# Autodesk Inventor assembly: Framework MASTER
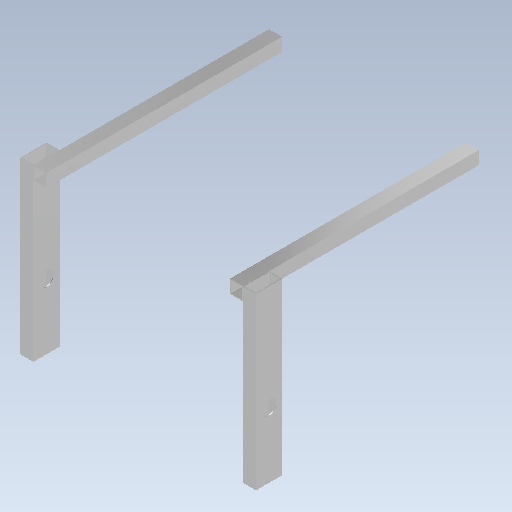
[picture p0: Inventor's stored thumbnail of the model, 512x512]
Saved by Autodesk Inventor 2020 (Build 240168000, 168)
## iProperties
Created: 2020-01-27
Part Number: Framework MASTER
Document SubType Name: Assembly
Designer: autum
Author: autum
## Documents named in this file (3)
- C:\Users\autum\Google Drive\Iron Riders 4180 (Roosevelt Robotics)\2019-2020\Build_Design\Robot 2020 (1)\Framework\Framework MASTER.iam
- C:\Users\autum\Google Drive\Iron Riders 4180 (Roosevelt Robotics)\2019-2020\Build_Design\Robot 2020 (1)\Framework\1x1 Top Frame.ipt
- C:\Users\autum\Google Drive\Iron Riders 4180 (Roosevelt Robotics)\2019-2020\Build_Design\Robot 2020 (1)\Framework\1x2 Frame.ipt
## Components (4 placed, 2 different names)
1. 1x1 Top Frame:1 — Mate:2, Flush:16, Flush:17
2. 1x1 Top Frame:2 — Flush:13, Flush:15, Mate:1
3. 1x2 Frame:1 — Flush:13, Flush:15, Mate:1
4. 1x2 Frame:2 — Mate:2, Flush:16, Flush:17
## Relationships (6: Flush 4, Mate 2)
- Flush:13: 1x1 Top Frame:2 ↔ 1x2 Frame:1
- Flush:15: 1x1 Top Frame:2 ↔ 1x2 Frame:1
- Mate:1: 1x1 Top Frame:2 ↔ 1x2 Frame:1
- Mate:2: 1x1 Top Frame:1 ↔ 1x2 Frame:2
- Flush:16: 1x1 Top Frame:1 ↔ 1x2 Frame:2
- Flush:17: 1x1 Top Frame:1 ↔ 1x2 Frame:2
